# Autodesk Inventor assembly: Assembly test
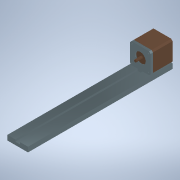
[picture p0: Inventor's stored thumbnail of the model, 180x180]
Saved by Autodesk Inventor 2021.2 (Build 252289000, 289)
## iProperties
Created: 2024-04-19
Part Number: Assembly test
Document SubType Name: Assembly
Designer: cioba
Author: cioba
## Documents named in this file (4)
- C:\Users\cioba\OneDrive\Desktop\syringe\Assembly test.iam
- C:\Users\cioba\OneDrive\Desktop\syringe\motor-01.ipt
- C:\Users\cioba\OneDrive\Desktop\syringe\attachment motor.ipt
- C:\Users\cioba\OneDrive\Desktop\syringe\sina.ipt
## Components (3 placed, 3 different names)
1. motor-01:1 — Rigid:1, Rigid:2
2. attachment motor:1 — Rigid:1
3. sina:1 — Rigid:2
## Relationships (2: WeldJoint 2)
- Rigid:1 [WeldJoint]: motor-01:1 ↔ attachment motor:1
- Rigid:2 [WeldJoint]: motor-01:1 ↔ sina:1
